# Autodesk Inventor assembly: top&cover
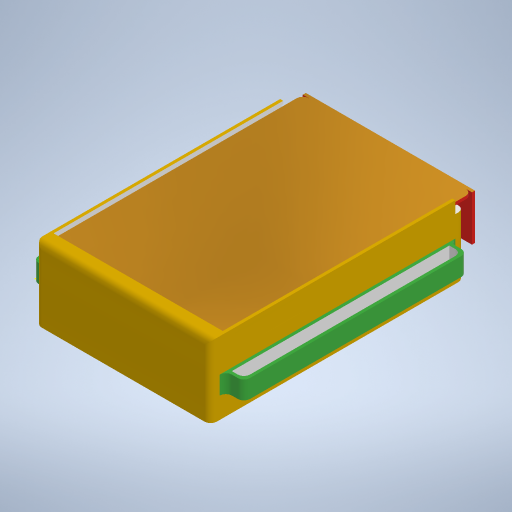
[picture p0: Inventor's stored thumbnail of the model, 512x512]
Saved by Autodesk Inventor 2023 (Build 270158000, 158)
## iProperties
Created: 2023-01-13
Part Number: top&cover
Document SubType Name: Assembly
Designer: zhanj390
Author: zhanj390
## Documents named in this file (3)
- C:\Users\zhanj390\Desktop\3P04_CAD_PM1_ZhangK\top&cover.iam
- C:\Users\zhanj390\Desktop\3P04_CAD_PM1_ZhangK\cover.ipt
- C:\Users\zhanj390\Desktop\3P04_CAD_PM1_ZhangK\top.ipt
## Components (2 placed, 2 different names)
1. top:1 — Mate:1, Mate:2, Mate:3, Mate:4
2. cover:1 — Mate:1, Mate:2, Mate:3, Mate:4
## Relationships (4: Mate 4)
- Mate:1: top:1 ↔ cover:1
- Mate:2: top:1 ↔ cover:1
- Mate:3: top:1 ↔ cover:1
- Mate:4: top:1 ↔ cover:1
